# Autodesk Inventor assembly: 2xSplitter
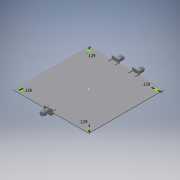
[picture p0: Inventor's stored thumbnail of the model, 180x180]
Saved by Autodesk Inventor 2018 (Build 220112000, 112)
## iProperties
Created: 2018-04-06
Part Number: 2xSplitter
Document SubType Name: Assembly
Designer: bbramman
Author: bbramman
## Documents named in this file (3)
- C:\Users\bbramman\OneDrive\Documents\Trapped Ion Research (Grad)\Electronics\pll-evalboard-synthesizer\Box CAD\2xSplitter.iam
- C:\Users\bbramman\OneDrive\Documents\Trapped Ion Research (Grad)\Electronics\pll-evalboard-synthesizer\Box CAD\2xSplitter.ipt
- C:\Users\bbramman\OneDrive\Documents\Trapped Ion Research (Grad)\Electronics\pll-evalboard-synthesizer\Box CAD\SMA-END.ipt
## Components (4 placed, 2 different names)
1. 2xSplitter:1 — Mate:1, Mate:2, Flush:1, Mate:3, Mate:4, Mate:5, Mate:6
2. SMA-END:1 — Mate:1, Mate:2, Flush:1
3. SMA-END:2 — Mate:3, Mate:4
4. SMA-END:3 — Mate:5, Mate:6
## Relationships (7: Mate 6, Flush 1)
- Mate:1: 2xSplitter:1 ↔ SMA-END:1
- Mate:2: 2xSplitter:1 ↔ SMA-END:1
- Flush:1 (48.26 mm): 2xSplitter:1 ↔ SMA-END:1
- Mate:3: 2xSplitter:1 ↔ SMA-END:2
- Mate:4: 2xSplitter:1 ↔ SMA-END:2
- Mate:5: 2xSplitter:1 ↔ SMA-END:3
- Mate:6: 2xSplitter:1 ↔ SMA-END:3
